# Autodesk Inventor assembly: sensor_platform
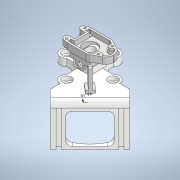
[picture p0: Inventor's stored thumbnail of the model, 180x180]
Saved by Autodesk Inventor 2022 (Build 260153070, 153G)
## iProperties
Created: 2021-06-08
Part Number: sensor_platform
Document SubType Name: Assembly
Designer: fraaw
Author: fraaw
## Documents named in this file (4)
- D:\repos\fingerSense\CAD\sensor_platform.iam
- D:\repos\fingerSense\CAD\franka_connector.ipt
- D:\repos\fingerSense\CAD\finger_mount.ipt
- D:\repos\fingerSense\CAD\lavalier_holder.ipt
## Components (3 placed, 3 different names)
1. franka_connector:1 — Cylindrical:1, Mate:1, Mate:2, Mate:3
2. finger_mount:1 — Cylindrical:1, Mate:1
3. lavalier_holder:1 — Mate:2, Mate:3
## Relationships (4: Mate 3, CylindricalJoint 1)
- Cylindrical:1: franka_connector:1 ↔ finger_mount:1
- Mate:1: franka_connector:1 ↔ finger_mount:1
- Mate:2: franka_connector:1 ↔ lavalier_holder:1
- Mate:3: franka_connector:1 ↔ lavalier_holder:1
